# Autodesk Inventor assembly: 컨버터 하우징
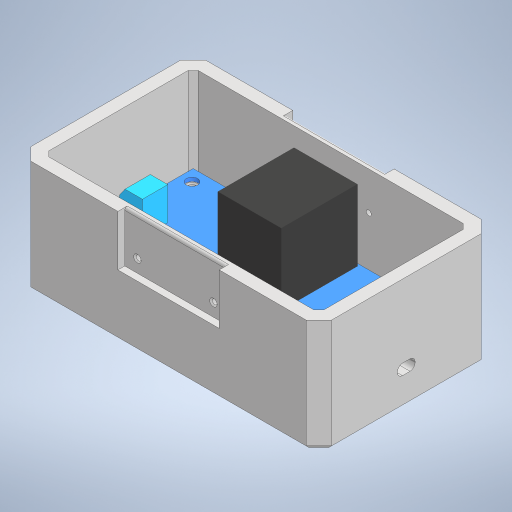
[picture p0: Inventor's stored thumbnail of the model, 512x512]
Saved by Autodesk Inventor 2023 (Build 270158000, 158)
## iProperties
Created: 2022-08-19
Part Number: 컨버터 하우징
Document SubType Name: Assembly
Designer: user
Author: user
## Documents named in this file (3)
- C:\Users\user\Desktop\PAI\PAI설계\전원 컨버터\컨버터 하우징.iam
- C:\Users\user\Desktop\PAI\PAI설계\범용 부품\AC-DC컨버터.ipt
- C:\Users\user\Desktop\PAI\PAI설계\전원 컨버터\컨버터 하우징.ipt
## Components (2 placed, 2 different names)
1. AC-DC컨버터:1 — 삽입:1, 삽입:2
2. 컨버터 하우징:1 — 삽입:1, 삽입:2
## Relationships (2: Insert 2)
- 삽입:1 [Insert]: AC-DC컨버터:1 ↔ 컨버터 하우징:1
- 삽입:2 [Insert]: AC-DC컨버터:1 ↔ 컨버터 하우징:1
